# Autodesk Inventor assembly: Neo with hexshaft
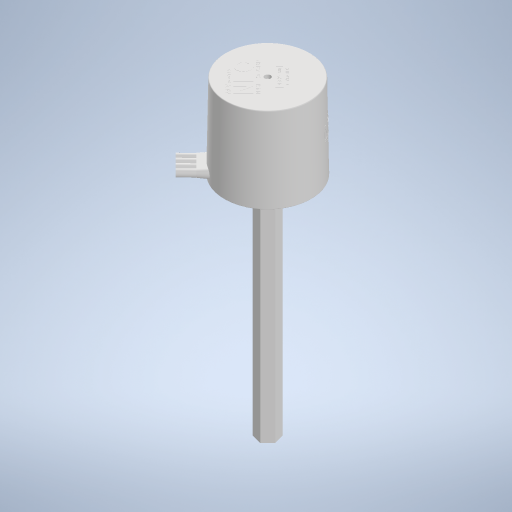
[picture p0: Inventor's stored thumbnail of the model, 512x512]
Saved by Autodesk Inventor 2024.1 (Build 281209000, 209)
## iProperties
Created: 2024-01-19
Part Number: Neo with hexshaft
Document SubType Name: Assembly
Designer: ey6
Author: ey6
## Documents named in this file (3)
- C:\Users\ey6\Documents\GitHub\Code-Red-2024-Cad\Neo with hexshaft.iam
- C:\Users\ey6\Downloads\REV-21-1650-V1.1\REV-21-1650-V1.1.ipt
- C:\Users\ey6\Downloads\Hexshaft 6 in.ipt
## Components (2 placed, 2 different names)
1. REV-21-1650-V1.1:1 — Mate:1, Mate:2, Insert:1
2. Hexshaft 6 in:1 — Mate:1, Mate:2, Insert:1
## Relationships (3: Mate 2, Insert 1)
- Mate:1: REV-21-1650-V1.1:1 ↔ Hexshaft 6 in:1
- Mate:2: REV-21-1650-V1.1:1 ↔ Hexshaft 6 in:1
- Insert:1: REV-21-1650-V1.1:1 ↔ Hexshaft 6 in:1
